# Autodesk Inventor assembly: DIL8-Socket+Package
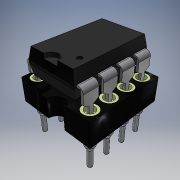
[picture p0: Inventor's stored thumbnail of the model, 180x180]
Saved by Autodesk Inventor 2018 (Build 220112000, 112)
## iProperties
Created: 2020-04-20
Part Number: DIL8-Socket+Package
Material: Všeobecné
Document SubType Name: Assembly
Designer: Jozko Mrkvicka
Author: Jozko Mrkvicka
## Documents named in this file (3)
- F:\Workspace\Projekty\Library\DIL8-Socket+Package.iam
- F:\Workspace\Projekty\Library\DIL8-Package.ipt
- F:\Workspace\Projekty\Library\DIL8-Socket.ipt
## Components (2 placed, 2 different names)
1. DIL8-Package:1 — Vložit:1, Proti sobě:1, Stejný směr:1
2. DIL8-Socket:1 — Vložit:1, Proti sobě:1, Proti sobě:2
## Relationships (4: Mate 2, Insert 1, Flush 1)
- Vložit:1 [Insert]: DIL8-Package:1 ↔ DIL8-Socket:1
- Proti sobě:1 [Mate]: DIL8-Package:1 ↔ DIL8-Socket:1
- Stejný směr:1 [Flush]: DIL8-Package:1
- Proti sobě:2 [Mate]: DIL8-Socket:1
